# Autodesk Inventor assembly: over bumper intake assembly
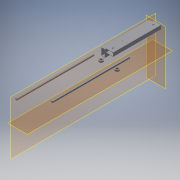
[picture p0: Inventor's stored thumbnail of the model, 180x180]
Saved by Autodesk Inventor 2018 (Build 220112000, 112)
## iProperties
Created: 2020-01-22
Part Number: over bumper intake assembly
Document SubType Name: Assembly
Designer: s-2513225
Author: s-2513225
## Documents named in this file (4)
- \\studenthome\students\S-2513225\GitHub\2020CAD\Over bumper intake\Assembly\over bumper intake assembly.iam
- \\studenthome\students\S-2513225\GitHub\2020CAD\Over bumper intake\Parts\arm.ipt
- \\studenthome\students\S-2513225\GitHub\2020CAD\Over bumper intake\Parts\hex shaft 1.ipt
- \\studenthome\students\S-2513225\GitHub\2020CAD\Over bumper intake\Parts\0_500_Hex_ID_x_1_125_OD_x_0_313_WD_Flanged_Bearing_v2_217-3875.ipt
## Components (6 placed, 3 different names)
1. arm:1 — Mate:3
2. hex shaft 1:1
3. arm:2 — Mate:1, Mate:2
4. hex shaft 1:2
5. 0_500_Hex_ID_x_1_125_OD_x_0_313_WD_Flanged_Bearing_v2_217-3875:1
6. 0_500_Hex_ID_x_1_125_OD_x_0_313_WD_Flanged_Bearing_v2_217-3875:2
## Relationships (3: Mate 3)
- Mate:1: arm:2
- Mate:2: arm:2
- Mate:3: arm:1
